# Autodesk Inventor assembly: Assembly - ElectromagnetGantryPlate V1
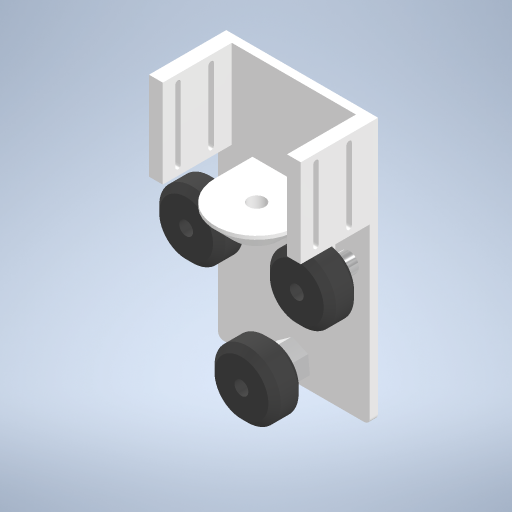
[picture p0: Inventor's stored thumbnail of the model, 512x512]
Saved by Autodesk Inventor 2023.2 (Build 272271030, 271C)
## iProperties
Created: 2023-04-28
Part Number: Assembly - ElectromagnetGantryPlate V1
Document SubType Name: Assembly
Designer: chase
Author: chase
## Documents named in this file (5)
- C:\Users\chase\OneDrive\Documents\GitHub\WU-AutomaticChessboard\CAD\Assembly - ElectromagnetGantryPlate V1.iam
- C:\Users\chase\OneDrive\Documents\GitHub\WU-AutomaticChessboard\CAD\Electromagnet Gantry Plate.ipt
- C:\Users\chase\OneDrive\Documents\GitHub\WU-AutomaticChessboard\CAD\EccentricNut 5mmID 11mmHex.ipt
- C:\Users\chase\OneDrive\Documents\GitHub\WU-AutomaticChessboard\CAD\Spacer 5mmID 8mmOD.ipt
- C:\Users\chase\OneDrive\Documents\GitHub\WU-AutomaticChessboard\CAD\VSlot RollerWheel.ipt
## Components (7 placed, 4 different names)
1. Electromagnet Gantry Plate:1 — Mate:1, Mate:2, Mate:3, Cylindrical:1, Mate:5
2. EccentricNut 5mmID 11mmHex:1 — Mate:1, Mate:4, Mate:5
3. Spacer 5mmID 8mmOD:1 — Mate:2, Insert:1
4. Spacer 5mmID 8mmOD:2 — Mate:3, Insert:2
5. VSlot RollerWheel:1 — Insert:1
6. VSlot RollerWheel:2 — Insert:2
7. VSlot RollerWheel:3 — Cylindrical:1, Mate:4
## Relationships (8: Mate 5, Insert 2, CylindricalJoint 1)
- Mate:1: Electromagnet Gantry Plate:1 ↔ EccentricNut 5mmID 11mmHex:1
- Mate:2: Electromagnet Gantry Plate:1 ↔ Spacer 5mmID 8mmOD:1
- Mate:3: Electromagnet Gantry Plate:1 ↔ Spacer 5mmID 8mmOD:2
- Insert:1: Spacer 5mmID 8mmOD:1 ↔ VSlot RollerWheel:1
- Insert:2: Spacer 5mmID 8mmOD:2 ↔ VSlot RollerWheel:2
- Cylindrical:1: Electromagnet Gantry Plate:1 ↔ VSlot RollerWheel:3
- Mate:4: EccentricNut 5mmID 11mmHex:1 ↔ VSlot RollerWheel:3
- Mate:5: Electromagnet Gantry Plate:1 ↔ EccentricNut 5mmID 11mmHex:1
